# Autodesk Inventor assembly: Bonus assembly
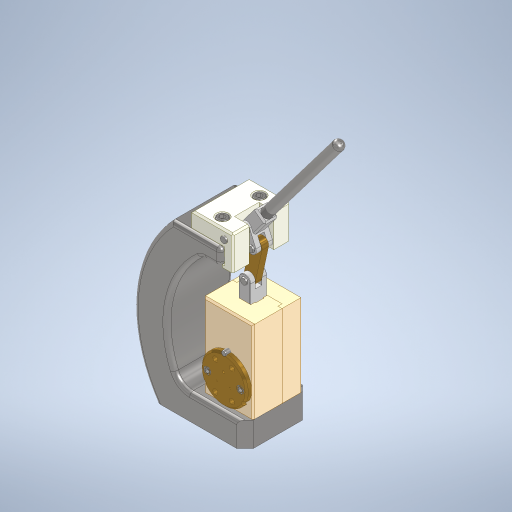
[picture p0: Inventor's stored thumbnail of the model, 512x512]
Saved by Autodesk Inventor 2024.1 (Build 281209000, 209)
## iProperties
Created: 2023-05-12
Part Number: Bonus assembly
Document SubType Name: Assembly
Designer: Raj
Author: Raj
## Documents named in this file (17)
- D:\New folder\Additional work\Bonus assembly.iam
- D:\New folder\Additional work\Gestell.ipt
- D:\New folder\Additional work\Schneidführung.ipt
- D:\New folder\Additional work\Schneidtrommel.ipt
- D:\New folder\Additional work\Part2.ipt
- D:\New folder\Additional work\Schneidstempel.ipt
- C:\Users\USER\OneDrive\Documents\Inventor\Content Center Files\R2024\en-US\BS EN 22 338  A - W\ISO 2338 - 8 m6 x 20 - ABS EN.ipt
- D:\New folder\Additional work\Hebel.ipt
- D:\New folder\Additional work\Kniehebel.ipt
- D:\New folder\Additional work\Lager.ipt
- C:\Users\USER\OneDrive\Documents\Inventor\Content Center Files\R2024\en-US\BS EN 22 338  A - W\ISO 2338 - 8 m6 x 70 - ABS EN.ipt
- D:\New folder\Additional work\Griff.ipt
- C:\Users\USER\OneDrive\Documents\Inventor\Content Center Files\R2024\en-US\ISO 4762(1)\DIN EN ISO 4762 - M8 x 20.ipt
- C:\Users\USER\OneDrive\Documents\Inventor\Content Center Files\R2024\en-US\ISO 2338  A - W\ISO 2338 - 6 m6 x 16 - A(1).ipt
- C:\Users\USER\OneDrive\Documents\Inventor\Content Center Files\R2024\en-US\ISO 4762(1)\DIN EN ISO 4762 - M6 x 16.ipt
- C:\Users\USER\OneDrive\Documents\Inventor\Content Center Files\R2024\en-US\ISO 4762(2)\ISO 4762 - M6 x 25ISO.ipt
- C:\Users\USER\OneDrive\Documents\Inventor\Content Center Files\R2024\en-US\ISO 4762(2)\ISO 4762 - M8 x 30ISO.ipt
## Components (27 placed, 16 different names)
1. Gestell:1 — Mate:1, Mate:2, Mate:3, Mate:7, Mate:8, Mate:9, Mate:20, Mate:21, Mate:22, Insert:12, Insert:13, Insert:14, Insert:15
2. Schneidführung:1 — Mate:1, Mate:2, Mate:3, Mate:4, Mate:5, Mate:6, Mate:10, Mate:11, Mate:26, Insert:4, Insert:5
3. Schneidtrommel:1 — Mate:4, Mate:5, Mate:6, Flush:28
4. Part2:1 — Mate:7, Mate:8, Mate:9, Insert:6, Insert:7, Insert:8, Insert:9, Insert:10, Insert:11
5. Schneidstempel:1 — Mate:10, Mate:11, Mate:12, Mate:13, Mate:15
6. BS EN 22338 A - withdrawn 8 m6 x 20 - A:1 — Mate:12, Mate:13, Mate:14
7. Hebel:1 — Mate:14, Mate:15, Mate:16, Mate:18
8. BS EN 22338 A - withdrawn 8 m6 x 20 - A:2 — Mate:16, Mate:17, Mate:19
9. Kniehebel:1 — Mate:17, Mate:18, Mate:19, Mate:25, Insert:1
10. Lager:1 — Mate:20, Mate:21, Mate:22, Mate:23, Mate:24, Insert:2, Insert:3
11. BS EN 22338 A - withdrawn 8 m6 x 70 - A:1 — Mate:23, Mate:24, Mate:25
12. Griff:1 — Insert:1
13. DIN EN ISO 4762 M8 x 20:1 — Insert:3
14. DIN EN ISO 4762 M8 x 20:2 — Insert:2
15. ISO 2338 A - withdrawn 6 m6 x 16 - A:1 — Mate:26, Flush:28
16. DIN EN ISO 4762 M6 x 16:1 — Insert:4
17. DIN EN ISO 4762 M6 x 16:2 — Insert:5
18. ISO 4762 M6 x 25:1 — Insert:6
19. ISO 4762 M6 x 25:2 — Insert:9
20. ISO 4762 M6 x 25:3 — Insert:7
21. ISO 4762 M6 x 25:4 — Insert:10
22. ISO 4762 M6 x 25:5 — Insert:8
23. ISO 4762 M6 x 25:6 — Insert:11
24. ISO 4762 M8 x 30:2 — Insert:12
25. ISO 4762 M8 x 30:3 — Insert:13
26. ISO 4762 M8 x 30:4 — Insert:14
27. ISO 4762 M8 x 30:5 — Insert:15
## Relationships (42: Mate 26, Insert 15, Flush 1)
- Mate:1: Gestell:1 ↔ Schneidführung:1
- Mate:2: Gestell:1 ↔ Schneidführung:1
- Mate:3: Gestell:1 ↔ Schneidführung:1
- Mate:4: Schneidführung:1 ↔ Schneidtrommel:1
- Mate:5: Schneidführung:1 ↔ Schneidtrommel:1
- Mate:6: Schneidführung:1 ↔ Schneidtrommel:1
- Mate:7: Gestell:1 ↔ Part2:1
- Mate:8: Gestell:1 ↔ Part2:1
- Mate:9: Gestell:1 ↔ Part2:1
- Mate:10: Schneidführung:1 ↔ Schneidstempel:1
- Mate:11: Schneidführung:1 ↔ Schneidstempel:1
- Mate:12: Schneidstempel:1 ↔ BS EN 22338 A - withdrawn 8 m6 x 20 - A:1
- Mate:13: Schneidstempel:1 ↔ BS EN 22338 A - withdrawn 8 m6 x 20 - A:1
- Mate:14: BS EN 22338 A - withdrawn 8 m6 x 20 - A:1 ↔ Hebel:1
- Mate:15: Schneidstempel:1 ↔ Hebel:1
- Mate:16: Hebel:1 ↔ BS EN 22338 A - withdrawn 8 m6 x 20 - A:2
- Mate:17: BS EN 22338 A - withdrawn 8 m6 x 20 - A:2 ↔ Kniehebel:1
- Mate:18: Hebel:1 ↔ Kniehebel:1
- Mate:19: BS EN 22338 A - withdrawn 8 m6 x 20 - A:2 ↔ Kniehebel:1
- Mate:20: Gestell:1 ↔ Lager:1
- Mate:21: Gestell:1 ↔ Lager:1
- Mate:22: Gestell:1 ↔ Lager:1
- Mate:23: Lager:1 ↔ BS EN 22338 A - withdrawn 8 m6 x 70 - A:1
- Mate:24: Lager:1 ↔ BS EN 22338 A - withdrawn 8 m6 x 70 - A:1
- Mate:25: Kniehebel:1 ↔ BS EN 22338 A - withdrawn 8 m6 x 70 - A:1
- Insert:1: Kniehebel:1 ↔ Griff:1
- Insert:2: Lager:1 ↔ DIN EN ISO 4762 M8 x 20:2
- Insert:3: Lager:1 ↔ DIN EN ISO 4762 M8 x 20:1
- Mate:26: Schneidführung:1 ↔ ISO 2338 A - withdrawn 6 m6 x 16 - A:1
- Flush:28: Schneidtrommel:1 ↔ ISO 2338 A - withdrawn 6 m6 x 16 - A:1
- Insert:4: Schneidführung:1 ↔ DIN EN ISO 4762 M6 x 16:1
- Insert:5: Schneidführung:1 ↔ DIN EN ISO 4762 M6 x 16:2
- Insert:6: Part2:1 ↔ ISO 4762 M6 x 25:1
- Insert:7: Part2:1 ↔ ISO 4762 M6 x 25:3
- Insert:8: Part2:1 ↔ ISO 4762 M6 x 25:5
- Insert:9: Part2:1 ↔ ISO 4762 M6 x 25:2
- Insert:10: Part2:1 ↔ ISO 4762 M6 x 25:4
- Insert:11: Part2:1 ↔ ISO 4762 M6 x 25:6
- Insert:12: Gestell:1 ↔ ISO 4762 M8 x 30:2
- Insert:13: Gestell:1 ↔ ISO 4762 M8 x 30:3
- Insert:14: Gestell:1 ↔ ISO 4762 M8 x 30:4
- Insert:15: Gestell:1 ↔ ISO 4762 M8 x 30:5
